# Autodesk Inventor assembly: Structure
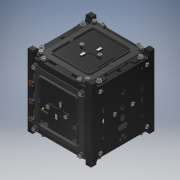
[picture p0: Inventor's stored thumbnail of the model, 180x180]
Saved by Autodesk Inventor 2018 (Build 220112000, 112)
## iProperties
Created: 2019-03-30
Part Number: Structure
Document SubType Name: Assembly
Designer: Bradley
Author: Bradley
## Documents named in this file (18)
- C:\Users\Bradley\Documents\GitHub\CougSat1-Hardware\CougSat1-Structure\CADModel\Imported\Structure.iam
- C:\Users\Bradley\Documents\GitHub\CougSat1-Hardware\CougSat1-Structure\CADModel\Imported\Structure_+X.ipt
- C:\Users\Bradley\Documents\GitHub\CougSat1-Hardware\CougSat1-Structure\CADModel\Imported\Structure_-X.ipt
- C:\Users\Bradley\Documents\GitHub\CougSat1-Hardware\CougSat1-Structure\CADModel\Imported\Structure_Y.ipt
- C:\Users\Bradley\Documents\GitHub\CougSat1-Hardware\CougSat1-Structure\CADModel\Imported\Structure_-Z.ipt
- C:\Users\Bradley\Documents\GitHub\CougSat1-Hardware\CougSat1-Structure\CADModel\Imported\Structure_SolarPanelHeatsink.ipt
- C:\Users\Bradley\Documents\GitHub\CougSat1-Hardware\CougSat1-Structure\CADModel\Imported\Structure_MagnetorquerForm.ipt
- C:\Users\Bradley\Documents\GitHub\Resources\SupplierDocuments\48 - Hardware\48-0361\48-0361.ipt
- C:\Users\Bradley\Documents\GitHub\Resources\SupplierDocuments\48 - Hardware\48-0340\48-0340.ipt
- C:\Users\Bradley\Documents\GitHub\Resources\SupplierDocuments\48 - Hardware\48-0350\48-0350.ipt
- C:\Users\Bradley\Documents\GitHub\Resources\SupplierDocuments\48 - Hardware\48-0300\48-0300.ipt
- C:\Users\Bradley\Documents\GitHub\Resources\SupplierDocuments\48 - Hardware\48-0001\48-0001.ipt
- C:\Users\Bradley\Documents\GitHub\Resources\SupplierDocuments\48 - Hardware\48-0381\48-0381.ipt
- C:\Users\Bradley\Documents\GitHub\Resources\SupplierDocuments\48 - Hardware\48-0362\48-0362.ipt
- C:\Users\Bradley\Documents\GitHub\Resources\SupplierDocuments\48 - Hardware\48-03A1\48-03A1.ipt
- C:\Users\Bradley\Documents\GitHub\Resources\SupplierDocuments\49 - Electromechanical\49-0006\49-0006.ipt
- C:\Users\Bradley\Documents\GitHub\Resources\SupplierDocuments\48 - Hardware\48-0280\48-0280.ipt
- C:\Users\Bradley\Documents\GitHub\CougSat1-Hardware\CougSat1-Payload\CADModel\Imported\Germination.iam
## Components (86 placed, 17 different names)
1. 48-0280:6 — Insert:143
2. 48-0280:5 — Insert:144
3. 48-0280:4 — Insert:145
4. 48-0280:3 — Insert:146
5. 48-0280:2 — Insert:147
6. 48-0280:1 — Insert:148
7. 49-0006:3 — Insert:138, Angle:3, Insert:143
8. 49-0006:2 — Insert:137, Angle:1, Insert:147
9. 49-0006:1 — Insert:139, Angle:2, Insert:145
10. 48-0001:1 — Insert:27
11. 48-0001:2 — Insert:140
12. 48-0300:1 — Insert:29, Insert:159
13. 48-0300:10 — Insert:156
14. 48-0300:11 — Insert:160
15. 48-0300:12 — Insert:54
16. 48-0300:2 — Insert:53
17. 48-0300:3 — Insert:51
18. 48-0300:4 — Insert:52
19. 48-0300:5 — Insert:83, Insert:87
20. 48-0300:6 — Insert:84, Insert:88
21. 48-0300:7 — Insert:85, Insert:90
22. 48-0300:8 — Insert:86, Insert:89
23. 48-0300:9 — Insert:153
24. 48-0340:1 — Insert:77
25. 48-0340:10 — Insert:90
26. 48-0340:2 — Insert:89
27. 48-0340:3 — Insert:78
28. 48-0340:4 — Insert:79
29. 48-0340:5 — Insert:80
30. 48-0340:6 — Insert:81
31. 48-0340:7 — Insert:82
32. 48-0340:8 — Insert:87
33. 48-0340:9 — Insert:88
34. 48-0350:1 — Insert:157
35. 48-0350:2 — Insert:158
36. 48-0350:3 — Insert:161
37. 48-0350:4 — Insert:162
38. 48-0350:5 — Insert:58
39. 48-0350:6 — Insert:57
40. 48-0350:7 — Insert:55
41. 48-0350:8 — Insert:56
42. 48-0362:1 — Insert:91
43. 48-0362:2 — Insert:92
44. 48-0362:3 — Insert:94
45. 48-0362:4 — Insert:93
46. 48-0361:1 — Insert:29
47. 48-0361:2
48. 48-0361:3
49. 48-0361:4
50. 48-0361:5
51. 48-0361:6
52. 48-0361:7
53. 48-0361:8
54. 48-0381:1 — Insert:59
55. 48-0381:18 — Insert:75
56. 48-0381:2 — Insert:60
57. 48-0381:3 — Insert:63
58. 48-0381:4 — Insert:64
59. 48-0381:5 — Insert:61
60. 48-0381:6 — Insert:62
61. 48-0381:7 — Insert:65
62. 48-0381:8 — Insert:66
63. 48-0381:9 — Insert:67
64. 48-0381:10 — Insert:68
65. 48-0381:11 — Insert:69
66. 48-0381:12 — Insert:70
67. 48-0381:13 — Insert:71
68. 48-0381:14 — Insert:72
69. 48-0381:15
70. 48-0381:16
71. 48-0381:17 — Insert:76
72. 48-03A1:1 — Insert:95
73. 48-03A1:2 — Insert:96
74. Structure_+X:1 — Mate:1, Mate:2, Mate:3, Insert:9, Insert:10, Insert:27, Insert:77, Insert:78, Insert:79, Insert:80, Insert:81, Insert:82, Insert:166
75. Structure_-X:1 — Insert:119, Insert:120, Insert:127, Insert:128, Insert:137, Insert:138, Insert:139, Angle:1, Angle:2, Angle:3, Insert:140, Insert:144, Insert:146, Insert:148, Insert:154, Insert:155
76. Structure_-Z:1 — Insert:9, Insert:10, Insert:51, Insert:52, Insert:53, Insert:54, Insert:55, Insert:56, Insert:57, Insert:58, Insert:83, Insert:84, Insert:85, Insert:86
77. Structure_MagnetorquerForm:1 — Insert:59, Insert:60, Insert:63, Insert:64, Insert:117, Insert:118
78. Structure_MagnetorquerForm:2 — Insert:91, Insert:92, Insert:93, Insert:94, Insert:119, Insert:120
79. Structure_MagnetorquerForm:3 — Insert:71, Insert:72, Insert:75, Insert:76, Insert:169, Insert:170
80. Structure_MagnetorquerForm:4 — Insert:65, Insert:66, Insert:69, Insert:70, Insert:121, Insert:122
81. Structure_SolarPanelHeatsink:2 — Insert:61, Insert:62, Insert:125, Insert:126
82. Structure_SolarPanelHeatsink:3 — Insert:95, Insert:96, Insert:127, Insert:128
83. Structure_SolarPanelHeatsink:4 — Insert:67, Insert:68, Insert:123, Insert:124
84. Structure_Y:1 — Insert:117, Insert:118, Insert:125, Insert:126, Insert:167, Insert:168
85. Structure_Y:2 — Insert:121, Insert:122, Insert:123, Insert:124, Insert:163
86. Germination:1 [sub-assembly] — Insert:153, Insert:154, Insert:155, Insert:156, Insert:157, Insert:158, Insert:159, Insert:160, Insert:161, Insert:162, Insert:163, Insert:166, Insert:167, Insert:168, Insert:169, Insert:170
## Relationships (103: Insert 97, Mate 3, Angle 3)
- Mate:1 (50 mm): Structure_+X:1
- Mate:2 (-49 mm): Structure_+X:1
- Mate:3 (50 mm): Structure_+X:1
- Insert:9: Structure_+X:1 ↔ Structure_-Z:1
- Insert:10: Structure_+X:1 ↔ Structure_-Z:1
- Insert:27: 48-0001:1 ↔ Structure_+X:1
- Insert:29: 48-0300:1 ↔ 48-0361:1
- [Insert]: 48-0300:9 ↔ 48-0361:5
- [Insert]: 48-0300:10 ↔ 48-0361:6
- [Insert]: 48-0300:11 ↔ 48-0361:7
- [Insert]: 48-0300:12 ↔ 48-0361:8
- [Insert]: 48-0300:2 ↔ 48-0361:2
- [Insert]: 48-0300:3 ↔ 48-0361:3
- [Insert]: 48-0300:4 ↔ 48-0361:4
- Insert:51: 48-0300:3 ↔ Structure_-Z:1
- Insert:52: 48-0300:4 ↔ Structure_-Z:1
- Insert:53: 48-0300:2 ↔ Structure_-Z:1
- Insert:54: 48-0300:12 ↔ Structure_-Z:1
- Insert:55: 48-0350:7 ↔ Structure_-Z:1
- Insert:56: 48-0350:8 ↔ Structure_-Z:1
- Insert:57: 48-0350:6 ↔ Structure_-Z:1
- Insert:58: 48-0350:5 ↔ Structure_-Z:1
- Insert:59 (1 mm): 48-0381:1 ↔ Structure_MagnetorquerForm:1
- Insert:60 (1 mm): 48-0381:2 ↔ Structure_MagnetorquerForm:1
- Insert:61 (1 mm): 48-0381:5 ↔ Structure_SolarPanelHeatsink:2
- Insert:62 (1 mm): 48-0381:6 ↔ Structure_SolarPanelHeatsink:2
- Insert:63 (1 mm): 48-0381:3 ↔ Structure_MagnetorquerForm:1
- Insert:64 (1 mm): 48-0381:4 ↔ Structure_MagnetorquerForm:1
- Insert:65 (1 mm): 48-0381:7 ↔ Structure_MagnetorquerForm:4
- Insert:66 (1 mm): 48-0381:8 ↔ Structure_MagnetorquerForm:4
- Insert:67 (1 mm): 48-0381:9 ↔ Structure_SolarPanelHeatsink:4
- Insert:68 (1 mm): 48-0381:10 ↔ Structure_SolarPanelHeatsink:4
- Insert:69 (1 mm): 48-0381:11 ↔ Structure_MagnetorquerForm:4
- Insert:70 (1 mm): 48-0381:12 ↔ Structure_MagnetorquerForm:4
- Insert:71 (1 mm): 48-0381:13 ↔ Structure_MagnetorquerForm:3
- Insert:72 (1 mm): 48-0381:14 ↔ Structure_MagnetorquerForm:3
- Insert:75 (1 mm): 48-0381:18 ↔ Structure_MagnetorquerForm:3
- Insert:76 (1 mm): 48-0381:17 ↔ Structure_MagnetorquerForm:3
- Insert:77 (1 mm): 48-0340:1 ↔ Structure_+X:1
- Insert:78 (1 mm): 48-0340:3 ↔ Structure_+X:1
- Insert:79 (1 mm): 48-0340:4 ↔ Structure_+X:1
- Insert:80 (1 mm): 48-0340:5 ↔ Structure_+X:1
- Insert:81 (1 mm): 48-0340:6 ↔ Structure_+X:1
- Insert:82 (1 mm): 48-0340:7 ↔ Structure_+X:1
- Insert:83: 48-0300:5 ↔ Structure_-Z:1
- Insert:84: 48-0300:6 ↔ Structure_-Z:1
- Insert:85: 48-0300:7 ↔ Structure_-Z:1
- Insert:86: 48-0300:8 ↔ Structure_-Z:1
- Insert:87 (1 mm): 48-0300:5 ↔ 48-0340:8
- Insert:88 (1 mm): 48-0300:6 ↔ 48-0340:9
- Insert:89 (1 mm): 48-0300:8 ↔ 48-0340:2
- Insert:90 (1 mm): 48-0300:7 ↔ 48-0340:10
- Insert:91 (1 mm): 48-0362:1 ↔ Structure_MagnetorquerForm:2
- Insert:92 (1 mm): 48-0362:2 ↔ Structure_MagnetorquerForm:2
- Insert:93 (1 mm): 48-0362:4 ↔ Structure_MagnetorquerForm:2
- Insert:94 (1 mm): 48-0362:3 ↔ Structure_MagnetorquerForm:2
- Insert:95 (1 mm): 48-03A1:1 ↔ Structure_SolarPanelHeatsink:3
- Insert:96 (1 mm): 48-03A1:2 ↔ Structure_SolarPanelHeatsink:3
- Insert:117: Structure_MagnetorquerForm:1 ↔ Structure_Y:1
- Insert:118: Structure_MagnetorquerForm:1 ↔ Structure_Y:1
- Insert:119: Structure_-X:1 ↔ Structure_MagnetorquerForm:2
- Insert:120: Structure_-X:1 ↔ Structure_MagnetorquerForm:2
- Insert:121: Structure_MagnetorquerForm:4 ↔ Structure_Y:2
- Insert:122: Structure_MagnetorquerForm:4 ↔ Structure_Y:2
- Insert:123: Structure_SolarPanelHeatsink:4 ↔ Structure_Y:2
- Insert:124: Structure_SolarPanelHeatsink:4 ↔ Structure_Y:2
- Insert:125: Structure_SolarPanelHeatsink:2 ↔ Structure_Y:1
- Insert:126: Structure_SolarPanelHeatsink:2 ↔ Structure_Y:1
- Insert:127: Structure_-X:1 ↔ Structure_SolarPanelHeatsink:3
- Insert:128: Structure_-X:1 ↔ Structure_SolarPanelHeatsink:3
- Insert:137: 49-0006:2 ↔ Structure_-X:1
- Insert:138: 49-0006:3 ↔ Structure_-X:1
- Insert:139: 49-0006:1 ↔ Structure_-X:1
- Angle:1 (0 deg): 49-0006:2 ↔ Structure_-X:1
- Angle:2 (0 deg): 49-0006:1 ↔ Structure_-X:1
- Angle:3 (0 deg): 49-0006:3 ↔ Structure_-X:1
- Insert:140: 48-0001:2 ↔ Structure_-X:1
- [Insert] (1 mm): 48-0381:16 ↔ Germination:1
- [Insert] (1 mm): 48-0381:15 ↔ Germination:1
- Insert:143: 48-0280:6 ↔ 49-0006:3
- Insert:144 (6.4 mm): 48-0280:5 ↔ Structure_-X:1
- Insert:145: 48-0280:4 ↔ 49-0006:1
- Insert:146 (6.4 mm): 48-0280:3 ↔ Structure_-X:1
- Insert:147: 48-0280:2 ↔ 49-0006:2
- Insert:148 (6.4 mm): 48-0280:1 ↔ Structure_-X:1
- Insert:153: 48-0300:9 ↔ Germination:1
- Insert:154: Structure_-X:1 ↔ Germination:1
- Insert:155: Structure_-X:1 ↔ Germination:1
- Insert:156: 48-0300:10 ↔ Germination:1
- Insert:157: 48-0350:1 ↔ Germination:1
- Insert:158: 48-0350:2 ↔ Germination:1
- Insert:159: 48-0300:1 ↔ Germination:1
- Insert:160: 48-0300:11 ↔ Germination:1
- Insert:161: 48-0350:3 ↔ Germination:1
- Insert:162: 48-0350:4 ↔ Germination:1
- Insert:163: Structure_Y:2 ↔ Germination:1
- [Insert]: Structure_Y:2 ↔ Germination:1
- [Insert]: Structure_+X:1 ↔ Germination:1
- Insert:166: Structure_+X:1 ↔ Germination:1
- Insert:167: Structure_Y:1 ↔ Germination:1
- Insert:168: Structure_Y:1 ↔ Germination:1
- Insert:169: Structure_MagnetorquerForm:3 ↔ Germination:1
- Insert:170: Structure_MagnetorquerForm:3 ↔ Germination:1
## Named parameters: d36_d32 = 0 mm, d37_d32 = 0 mm, d40_d32 = 0 mm, d52_d32 = 0 mm, d53_d32 = 0 mm, d54_d32 = 0 mm, d55_d32 = 0 mm, SolarPanelThickness = 1 mm, PXThickness = 1 mm, NZThickness = 1 mm
